# Autodesk Inventor assembly: HINGE
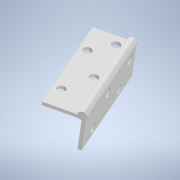
[picture p0: Inventor's stored thumbnail of the model, 180x180]
Saved by Autodesk Inventor 2021 (Build 250183000, 183)
## iProperties
Created: 2023-05-14
Part Number: HINGE
Document SubType Name: Assembly
Designer: Sahil Nadaf
Author: Sahil Nadaf
## Documents named in this file (3)
- D:\Engg exploration\HINGE.iam
- D:\Engg exploration\middle portion.ipt
- D:\Engg exploration\side part of hinge.ipt
## Components (3 placed, 2 different names)
1. middle portion:1 — Rigid:1, Rigid:2
2. side part of hinge:1 — Rigid:1
3. side part of hinge:2 — Rigid:2
## Relationships (2: WeldJoint 2)
- Rigid:1 [WeldJoint]: middle portion:1 ↔ side part of hinge:1
- Rigid:2 [WeldJoint]: middle portion:1 ↔ side part of hinge:2
